# Autodesk Inventor assembly: end_mould_base
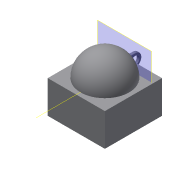
[picture p0: Inventor's stored thumbnail of the model, 180x180]
Saved by Autodesk Inventor 2017 (Build 210142000, 142)
## iProperties
Created: 2018-06-13
Part Number: end_mould_base
Document SubType Name: Assembly
Designer: Nic
Author: Nic
## Documents named in this file (3)
- C:\Users\Nic\Documents\Antenna\end_mould_base.iam
- C:\Users\Nic\Documents\Antenna\mould_casing.ipt
- C:\Users\Nic\Documents\Antenna\endmould_proc1.ipt
## Components (2 placed, 2 different names)
1. mould_casing:1 — Mate:1, Mate:2, Ball:1, Angle:1, Angle:2
2. endmould_proc1:1 — Ball:1, Angle:1, Angle:2
## Relationships (5: Mate 2, Angle 2, BallJoint 1)
- Mate:1: mould_casing:1
- Mate:2: mould_casing:1
- Ball:1: mould_casing:1 ↔ endmould_proc1:1
- Angle:1 (0 deg): mould_casing:1 ↔ endmould_proc1:1
- Angle:2 (0 deg): mould_casing:1 ↔ endmould_proc1:1
